# Autodesk Inventor assembly: FarmBot
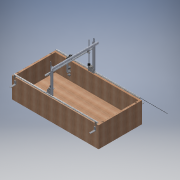
[picture p0: Inventor's stored thumbnail of the model, 180x180]
Saved by Autodesk Inventor 2017 (Build 210142000, 142)
## iProperties
Created: 2016-12-12
Part Number: FarmBot
Document SubType Name: Assembly
Designer: umr
Author: umr
## Documents named in this file (9)
- D:\SeniorProject\Models2\FarmBot.iam
- D:\SeniorProject\Models2\BedAssembly\BedAseembly.iam
- D:\SeniorProject\Models2\Case\Case.iam
- D:\SeniorProject\Models2\LED Structure\LED Structure Assembly.iam
- D:\SeniorProject\Models2\Gantry\GantryDown.iam
- D:\SeniorProject\Models2\BeltMain.ipt
- D:\SeniorProject\Models2\Gantry\GantryUp.iam
- D:\SeniorProject\Models2\30x60SigmaLong.ipt
- D:\SeniorProject\Models2\Gantry\GantryDown_MIR1.iam
## Components (8 placed, 8 different names)
1. BedAseembly:2 [sub-assembly] — Mate:10, Mate:11, Mate:12, Mate:13, Mate:14, Mate:15, Mate:16, Mate:19, Mate:20, Tangent:1, Tangent:3, Mate:21
2. Case:1 [sub-assembly] — Mate:10, Mate:11, Mate:12, Mate:13
3. LED Structure Assembly:1 [sub-assembly] — Mate:14, Mate:15, Mate:16
4. GantryDown:1 [sub-assembly] — Tangent:1, Tangent:2, Tangent:3, Mate:21, Mate:22, Mate:23, Mate:25, Flush:2, Flush:3, Flush:4
5. BeltMain:1 — Mate:19, Mate:20, Tangent:2
6. GantryUp:1 [sub-assembly] — Mate:22, Mate:23, Mate:26
7. 30x60SigmaLong:1 — Mate:25, Flush:2
8. GantryDown_MIR1:1 [sub-assembly] — Flush:3, Flush:4, Mate:26
## Relationships (20: Mate 14, Tangent 3, Flush 3)
- Mate:10: BedAseembly:2 ↔ Case:1
- Mate:11: BedAseembly:2 ↔ Case:1
- Mate:12: BedAseembly:2 ↔ Case:1
- Mate:13: BedAseembly:2 ↔ Case:1
- Mate:14: BedAseembly:2 ↔ LED Structure Assembly:1
- Mate:15: BedAseembly:2 ↔ LED Structure Assembly:1
- Mate:16: BedAseembly:2 ↔ LED Structure Assembly:1
- Mate:19: BedAseembly:2 ↔ BeltMain:1
- Mate:20 (3 mm): BedAseembly:2 ↔ BeltMain:1
- Tangent:1: BedAseembly:2 ↔ GantryDown:1
- Tangent:2: GantryDown:1 ↔ BeltMain:1
- Tangent:3: BedAseembly:2 ↔ GantryDown:1
- Mate:21: BedAseembly:2 ↔ GantryDown:1
- Mate:22: GantryDown:1 ↔ GantryUp:1
- Mate:23 (300 mm): GantryDown:1 ↔ GantryUp:1
- Mate:25: GantryDown:1 ↔ 30x60SigmaLong:1
- Flush:2: GantryDown:1 ↔ 30x60SigmaLong:1
- Flush:3: GantryDown:1 ↔ GantryDown_MIR1:1
- Flush:4: GantryDown:1 ↔ GantryDown_MIR1:1
- Mate:26: GantryUp:1 ↔ GantryDown_MIR1:1
